# Autodesk Inventor assembly: Transmission_MIR
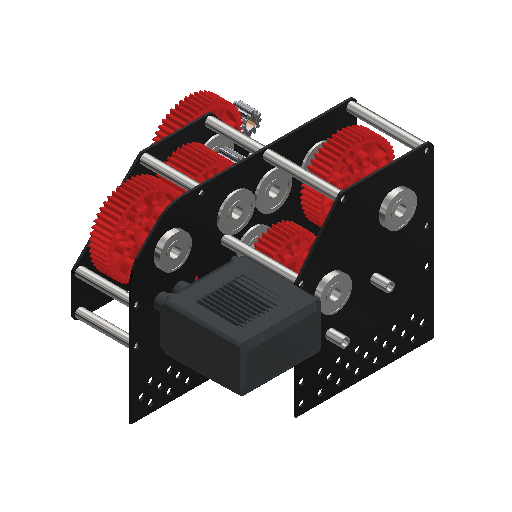
[picture p0: Inventor's stored thumbnail of the model, 512x512]
Saved by Autodesk Inventor 2024 (Build 280153000, 153)
## iProperties
Created: 2023-09-09
Part Number: Transmission_MIR
Document SubType Name: Assembly
Designer: aaron
Author: aaron
## Documents named in this file (14)
- C:\Users\aaron\Documents\Inventor\TritonRobotics\library\Stock Material\Plates\POM\Transmision\Transmission_MIR.iam
- C:\Users\aaron\Documents\Inventor\TritonRobotics\library\Stock Material\Plates\POM\Transmision\MainLayer_MIR.ipt
- C:\Users\aaron\Documents\Inventor\TritonRobotics\library\Stock Material\Plates\POM\Transmision\BottomLayer_MIR.ipt
- C:\Users\aaron\Documents\Inventor\TritonRobotics\library\Stock Material\Plates\POM\Transmision\Top Layer_MIR.ipt
- C:\Users\aaron\Documents\Inventor\TritonRobotics\library\VEX Library\Structure\Metal Spacers\1.0 1-2 od_MIR3.ipt
- C:\Users\aaron\Documents\Inventor\TritonRobotics\library\VEX Library\Structure\Metal Spacers\0.25 1-2 od_MIR3.ipt
- C:\Users\aaron\Documents\Inventor\TritonRobotics\library\VEX Library\Motion\HS Shaft\bearing_MIR1.ipt
- C:\Users\aaron\Documents\Inventor\TritonRobotics\library\VEX Library\Subsystems\PTOS\PTO .5 v1.1_MIR.iam
- C:\Users\aaron\Documents\Inventor\TritonRobotics\library\VEX Library\Subsystems\PTOS\PTO 1 v1.1_MIR.iam
- C:\Users\aaron\Documents\Inventor\TritonRobotics\library\VEX Library\Electronics\V5 Motor_MIR6.ipt
- C:\Users\aaron\Documents\Inventor\TritonRobotics\library\VEX Library\Motion\Gears\High Strength\36 Tooth\36T High Strength Gear v2_MIR3.ipt
- C:\Users\aaron\Documents\Inventor\TritonRobotics\library\VEX Library\Motion\Gears\Low Strength\36T Gear_MIR.ipt
- C:\Users\aaron\Documents\Inventor\TritonRobotics\library\VEX Library\Motion\Gears\High Strength\48 Tooth\48 High Strength Gear V2_MIR2.ipt
- C:\Users\aaron\Documents\Inventor\TritonRobotics\library\VEX Library\Motion\Gears\High Strength\12 Tooth\HS 12T Gear, No Insert_MIR2.ipt
## Components (55 placed, 13 different names)
1. MainLayer_MIR:1 — Mate:6, Mate:4, Mate:3, Mate:5, Mate:2, Mate:1, Mate:26, Mate:25, Mate:48, Mate:31, Mate:50, Mate:49, Mate:54, Mate:53, Mate:56, Mate:55, Mate:52, Mate:51, Mate:62, Mate:61, Mate:68, Mate:67, Mate:70, Mate:69, Mate:72, Mate:71, Mate:74, Mate:73, Mate:76, Mate:75, Mate:89, Mate:88, Mate:87, Mate:92
2. BottomLayer_MIR:1 — Mate:6, Mate:4, Mate:3, Mate:78, Mate:77, Mate:80, Mate:79, Mate:82, Mate:81, Mate:84, Mate:83
3. Top Layer_MIR:1 — Mate:5, Mate:2, Mate:1, Mate:10, Mate:9, Mate:18, Mate:17, Mate:22, Mate:21, Mate:20, Mate:19, Mate:64, Mate:63, Mate:66, Mate:65, Mate:85, Mate:86
4. 1.0 1-2 od_MIR3:1 — Mate:8, Mate:7
5. 1.0 1-2 od_MIR3:2 — Mate:10, Mate:9, Mate:8, Mate:7
6. 1.0 1-2 od_MIR3:3 — Mate:18, Mate:17, Mate:12, Mate:11
7. 1.0 1-2 od_MIR3:4 — Mate:12, Mate:11
8. 1.0 1-2 od_MIR3:5 — Mate:22, Mate:21, Mate:14, Mate:13
9. 1.0 1-2 od_MIR3:6 — Mate:14, Mate:13
10. 1.0 1-2 od_MIR3:7 — Mate:20, Mate:19, Mate:16, Mate:15
11. 1.0 1-2 od_MIR3:8 — Mate:16, Mate:15
12. 1.0 1-2 od_MIR3:9 — Mate:26, Mate:24, Mate:23
13. 1.0 1-2 od_MIR3:10 — Mate:25, Mate:24, Mate:23
14. 1.0 1-2 od_MIR3:11 — Mate:30, Mate:29
15. 0.25 1-2 od_MIR3:1 — Mate:30, Mate:29, Mate:28, Mate:27
16. 0.25 1-2 od_MIR3:2 — Mate:48, Mate:31, Mate:28, Mate:27
17. 1.0 1-2 od_MIR3:12 — Mate:35, Mate:34
18. 0.25 1-2 od_MIR3:3 — Mate:50, Mate:35, Mate:34, Mate:33, Mate:32
19. 0.25 1-2 od_MIR3:4 — Mate:49, Mate:33, Mate:32
20. 1.0 1-2 od_MIR3:13 — Mate:54, Mate:53, Mate:39, Mate:38
21. 0.25 1-2 od_MIR3:5 — Mate:39, Mate:38, Mate:37, Mate:36
22. 0.25 1-2 od_MIR3:6 — Mate:37, Mate:36
23. 1.0 1-2 od_MIR3:14 — Mate:56, Mate:55, Mate:43, Mate:42
24. 0.25 1-2 od_MIR3:7 — Mate:43, Mate:42, Mate:41, Mate:40
25. 0.25 1-2 od_MIR3:8 — Mate:41, Mate:40
26. 1.0 1-2 od_MIR3:15 — Mate:52, Mate:51, Mate:47, Mate:46
27. 0.25 1-2 od_MIR3:9 — Mate:47, Mate:46, Mate:45, Mate:44
28. 0.25 1-2 od_MIR3:10 — Mate:45, Mate:44
29. 1.0 1-2 od_MIR3:16 — Mate:62, Mate:61, Mate:60, Mate:59
30. 0.25 1-2 od_MIR3:11 — Mate:60, Mate:59, Mate:58, Mate:57
31. 0.25 1-2 od_MIR3:12 — Mate:58, Mate:57
32. bearing_MIR1:1 — Mate:64, Mate:63
33. bearing_MIR1:2 — Mate:66, Mate:65
34. bearing_MIR1:3 — Mate:68, Mate:67, Mate:93, Mate:94
35. bearing_MIR1:4 — Mate:70, Mate:69, Mate:96
36. bearing_MIR1:5 — Mate:72, Mate:71, Mate:90, Mate:100
37. bearing_MIR1:6 — Mate:74, Mate:73
38. bearing_MIR1:7 — Mate:78, Mate:77
39. bearing_MIR1:8 — Mate:76, Mate:75, Mate:101
40. bearing_MIR1:9 — Mate:80, Mate:79
41. bearing_MIR1:10 — Mate:82, Mate:81, Mate:97
42. bearing_MIR1:11 — Mate:84, Mate:83, Mate:95
43. PTO .5 v1.1_MIR:1 [sub-assembly] — Mate:85
44. PTO 1 v1.1_MIR:1 [sub-assembly] — Mate:86
45. V5 Motor_MIR6:1 — Mate:89, Mate:88, Mate:87
46. 36T High Strength Gear v2_MIR3:1 — Mate:90
47. 36T Gear_MIR:1 — Mate:92
48. 48 High Strength Gear V2_MIR2:1 — Mate:93
49. HS 12T Gear, No Insert_MIR2:1 — Mate:94
50. 48 High Strength Gear V2_MIR2:2 — Mate:95
51. HS 12T Gear, No Insert_MIR2:2 — Mate:96
52. 36T High Strength Gear v2_MIR3:2 — Mate:97, Mate:99, Mate:98
53. 36T High Strength Gear v2_MIR3:3 — Mate:99, Mate:98
54. 36T Gear_MIR:2 — Mate:100
55. 48 High Strength Gear V2_MIR2:3 — Mate:101
## Relationships (100: Mate 100)
- Mate:6 (38.1 mm): MainLayer_MIR:1 ↔ BottomLayer_MIR:1
- Mate:4: MainLayer_MIR:1 ↔ BottomLayer_MIR:1
- Mate:3: MainLayer_MIR:1 ↔ BottomLayer_MIR:1
- Mate:5 (50.8 mm): MainLayer_MIR:1 ↔ Top Layer_MIR:1
- Mate:2: MainLayer_MIR:1 ↔ Top Layer_MIR:1
- Mate:1: MainLayer_MIR:1 ↔ Top Layer_MIR:1
- Mate:10: Top Layer_MIR:1 ↔ 1.0 1-2 od_MIR3:2
- Mate:9: Top Layer_MIR:1 ↔ 1.0 1-2 od_MIR3:2
- Mate:8: 1.0 1-2 od_MIR3:1 ↔ 1.0 1-2 od_MIR3:2
- Mate:7: 1.0 1-2 od_MIR3:1 ↔ 1.0 1-2 od_MIR3:2
- Mate:18: Top Layer_MIR:1 ↔ 1.0 1-2 od_MIR3:3
- Mate:17: Top Layer_MIR:1 ↔ 1.0 1-2 od_MIR3:3
- Mate:12: 1.0 1-2 od_MIR3:3 ↔ 1.0 1-2 od_MIR3:4
- Mate:11: 1.0 1-2 od_MIR3:3 ↔ 1.0 1-2 od_MIR3:4
- Mate:22: Top Layer_MIR:1 ↔ 1.0 1-2 od_MIR3:5
- Mate:21: Top Layer_MIR:1 ↔ 1.0 1-2 od_MIR3:5
- Mate:14: 1.0 1-2 od_MIR3:5 ↔ 1.0 1-2 od_MIR3:6
- Mate:13: 1.0 1-2 od_MIR3:5 ↔ 1.0 1-2 od_MIR3:6
- Mate:20: Top Layer_MIR:1 ↔ 1.0 1-2 od_MIR3:7
- Mate:19: Top Layer_MIR:1 ↔ 1.0 1-2 od_MIR3:7
- Mate:16: 1.0 1-2 od_MIR3:7 ↔ 1.0 1-2 od_MIR3:8
- Mate:15: 1.0 1-2 od_MIR3:7 ↔ 1.0 1-2 od_MIR3:8
- Mate:26: MainLayer_MIR:1 ↔ 1.0 1-2 od_MIR3:9
- Mate:25: MainLayer_MIR:1 ↔ 1.0 1-2 od_MIR3:10
- Mate:24: 1.0 1-2 od_MIR3:9 ↔ 1.0 1-2 od_MIR3:10
- Mate:23: 1.0 1-2 od_MIR3:9 ↔ 1.0 1-2 od_MIR3:10
- Mate:30: 1.0 1-2 od_MIR3:11 ↔ 0.25 1-2 od_MIR3:1
- Mate:29: 1.0 1-2 od_MIR3:11 ↔ 0.25 1-2 od_MIR3:1
- Mate:48: MainLayer_MIR:1 ↔ 0.25 1-2 od_MIR3:2
- Mate:31: MainLayer_MIR:1 ↔ 0.25 1-2 od_MIR3:2
- Mate:28: 0.25 1-2 od_MIR3:1 ↔ 0.25 1-2 od_MIR3:2
- Mate:27: 0.25 1-2 od_MIR3:1 ↔ 0.25 1-2 od_MIR3:2
- Mate:50: MainLayer_MIR:1 ↔ 0.25 1-2 od_MIR3:3
- Mate:35: 1.0 1-2 od_MIR3:12 ↔ 0.25 1-2 od_MIR3:3
- Mate:34: 1.0 1-2 od_MIR3:12 ↔ 0.25 1-2 od_MIR3:3
- Mate:49: MainLayer_MIR:1 ↔ 0.25 1-2 od_MIR3:4
- Mate:33: 0.25 1-2 od_MIR3:3 ↔ 0.25 1-2 od_MIR3:4
- Mate:32: 0.25 1-2 od_MIR3:3 ↔ 0.25 1-2 od_MIR3:4
- Mate:54: MainLayer_MIR:1 ↔ 1.0 1-2 od_MIR3:13
- Mate:53: MainLayer_MIR:1 ↔ 1.0 1-2 od_MIR3:13
- Mate:39: 1.0 1-2 od_MIR3:13 ↔ 0.25 1-2 od_MIR3:5
- Mate:38: 1.0 1-2 od_MIR3:13 ↔ 0.25 1-2 od_MIR3:5
- Mate:37: 0.25 1-2 od_MIR3:5 ↔ 0.25 1-2 od_MIR3:6
- Mate:36: 0.25 1-2 od_MIR3:5 ↔ 0.25 1-2 od_MIR3:6
- Mate:56: MainLayer_MIR:1 ↔ 1.0 1-2 od_MIR3:14
- Mate:55: MainLayer_MIR:1 ↔ 1.0 1-2 od_MIR3:14
- Mate:43: 1.0 1-2 od_MIR3:14 ↔ 0.25 1-2 od_MIR3:7
- Mate:42: 1.0 1-2 od_MIR3:14 ↔ 0.25 1-2 od_MIR3:7
- Mate:41: 0.25 1-2 od_MIR3:7 ↔ 0.25 1-2 od_MIR3:8
- Mate:40: 0.25 1-2 od_MIR3:7 ↔ 0.25 1-2 od_MIR3:8
- Mate:52: MainLayer_MIR:1 ↔ 1.0 1-2 od_MIR3:15
- Mate:51: MainLayer_MIR:1 ↔ 1.0 1-2 od_MIR3:15
- Mate:47: 1.0 1-2 od_MIR3:15 ↔ 0.25 1-2 od_MIR3:9
- Mate:46: 1.0 1-2 od_MIR3:15 ↔ 0.25 1-2 od_MIR3:9
- Mate:45: 0.25 1-2 od_MIR3:9 ↔ 0.25 1-2 od_MIR3:10
- Mate:44: 0.25 1-2 od_MIR3:9 ↔ 0.25 1-2 od_MIR3:10
- Mate:62: MainLayer_MIR:1 ↔ 1.0 1-2 od_MIR3:16
- Mate:61: MainLayer_MIR:1 ↔ 1.0 1-2 od_MIR3:16
- Mate:60: 1.0 1-2 od_MIR3:16 ↔ 0.25 1-2 od_MIR3:11
- Mate:59: 1.0 1-2 od_MIR3:16 ↔ 0.25 1-2 od_MIR3:11
- Mate:58: 0.25 1-2 od_MIR3:11 ↔ 0.25 1-2 od_MIR3:12
- Mate:57: 0.25 1-2 od_MIR3:11 ↔ 0.25 1-2 od_MIR3:12
- Mate:64: Top Layer_MIR:1 ↔ bearing_MIR1:1
- Mate:63: Top Layer_MIR:1 ↔ bearing_MIR1:1
- Mate:66: Top Layer_MIR:1 ↔ bearing_MIR1:2
- Mate:65: Top Layer_MIR:1 ↔ bearing_MIR1:2
- Mate:68: MainLayer_MIR:1 ↔ bearing_MIR1:3
- Mate:67: MainLayer_MIR:1 ↔ bearing_MIR1:3
- Mate:70: MainLayer_MIR:1 ↔ bearing_MIR1:4
- Mate:69: MainLayer_MIR:1 ↔ bearing_MIR1:4
- Mate:72: MainLayer_MIR:1 ↔ bearing_MIR1:5
- Mate:71: MainLayer_MIR:1 ↔ bearing_MIR1:5
- Mate:74: MainLayer_MIR:1 ↔ bearing_MIR1:6
- Mate:73: MainLayer_MIR:1 ↔ bearing_MIR1:6
- Mate:78: BottomLayer_MIR:1 ↔ bearing_MIR1:7
- Mate:77: BottomLayer_MIR:1 ↔ bearing_MIR1:7
- Mate:76: MainLayer_MIR:1 ↔ bearing_MIR1:8
- Mate:75: MainLayer_MIR:1 ↔ bearing_MIR1:8
- Mate:80: BottomLayer_MIR:1 ↔ bearing_MIR1:9
- Mate:79: BottomLayer_MIR:1 ↔ bearing_MIR1:9
- Mate:82: BottomLayer_MIR:1 ↔ bearing_MIR1:10
- Mate:81: BottomLayer_MIR:1 ↔ bearing_MIR1:10
- Mate:84: BottomLayer_MIR:1 ↔ bearing_MIR1:11
- Mate:83: BottomLayer_MIR:1 ↔ bearing_MIR1:11
- Mate:85: Top Layer_MIR:1 ↔ PTO .5 v1.1_MIR:1
- Mate:86: Top Layer_MIR:1 ↔ PTO 1 v1.1_MIR:1
- Mate:89: MainLayer_MIR:1 ↔ V5 Motor_MIR6:1
- Mate:88: MainLayer_MIR:1 ↔ V5 Motor_MIR6:1
- Mate:87: MainLayer_MIR:1 ↔ V5 Motor_MIR6:1
- Mate:90: bearing_MIR1:5 ↔ 36T High Strength Gear v2_MIR3:1
- Mate:92: MainLayer_MIR:1 ↔ 36T Gear_MIR:1
- Mate:93: bearing_MIR1:3 ↔ 48 High Strength Gear V2_MIR2:1
- Mate:94: bearing_MIR1:3 ↔ HS 12T Gear, No Insert_MIR2:1
- Mate:95: bearing_MIR1:11 ↔ 48 High Strength Gear V2_MIR2:2
- Mate:96: bearing_MIR1:4 ↔ HS 12T Gear, No Insert_MIR2:2
- Mate:97: bearing_MIR1:10 ↔ 36T High Strength Gear v2_MIR3:2
- Mate:99: 36T High Strength Gear v2_MIR3:2 ↔ 36T High Strength Gear v2_MIR3:3
- Mate:98: 36T High Strength Gear v2_MIR3:2 ↔ 36T High Strength Gear v2_MIR3:3
- Mate:100: bearing_MIR1:5 ↔ 36T Gear_MIR:2
- Mate:101: bearing_MIR1:8 ↔ 48 High Strength Gear V2_MIR2:3
